# Autodesk Inventor assembly: PCB_Housing
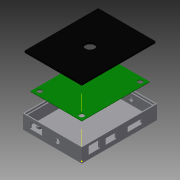
[picture p0: Inventor's stored thumbnail of the model, 180x180]
Saved by Autodesk Inventor 2015 (Build 190159000, 159)
## iProperties
Created: 2015-02-12
Part Number: PCB_Housing
Document SubType Name: Assembly
Designer: 477grp12
Mass: 27.5778 g
Surface Area: 356.467 cm^2
Volume: 27.5778 cm^3
Density: 1 g/cm^3
Author: 477grp12
## Documents named in this file (4)
- N:\bike-hud\MODELS\HelmetHUD\PCB_Housing.iam
- N:\bike-hud\MODELS\HelmetHUD\mainPCB.ipt
- N:\bike-hud\MODELS\HelmetHUD\pcbProtectiveCase.ipt
- N:\bike-hud\MODELS\HelmetHUD\pcbProtectiveCaseTop.ipt
## Components (3 placed, 3 different names)
1. mainPCB:1 — Mate:1, Mate:3, Mate:10
2. pcbProtectiveCase:1 — Mate:2, Mate:4, Mate:8, Mate:11
3. pcbProtectiveCaseTop:1 — Mate:5, Mate:7
## Relationships (12: Mate 12)
- Mate:1: mainPCB:1
- Mate:2: pcbProtectiveCase:1
- Mate:3: mainPCB:1
- Mate:4: pcbProtectiveCase:1
- Mate:5: pcbProtectiveCaseTop:1
- Mate:6
- Mate:7: pcbProtectiveCaseTop:1
- Mate:8: pcbProtectiveCase:1
- Mate:9
- Mate:10: mainPCB:1
- Mate:11: pcbProtectiveCase:1
- Mate:12
